# Autodesk Inventor assembly: ude_MIR
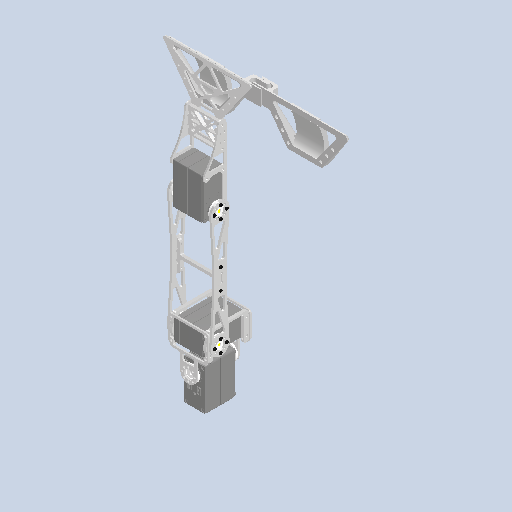
[picture p0: Inventor's stored thumbnail of the model, 512x512]
Saved by Autodesk Inventor 2024 (Build 280153000, 153)
## iProperties
Created: 2023-03-29
Part Number: ude_MIR
Document SubType Name: Assembly
Designer: right
Mass: 126.683 g
Surface Area: 569.35 cm^2
Volume: 110.135 cm^3
Density: 1.15025 g/cm^3
Author: right
## Documents named in this file (10)
- C:\Users\right\OneDrive\ドキュメント\Inventor\V2二足Light＿仮\ude_MIR.iam
- C:\Users\right\OneDrive\ドキュメント\Inventor\V2二足Light＿仮\KRS2500_scale_MIR1.ipt
- C:\Users\right\OneDrive\ドキュメント\Inventor\V2二足Light＿仮\02157_SmallDiameterHornB_MIR1.ipt
- C:\Users\right\OneDrive\ドキュメント\Inventor\V2二足Light＿仮\kata_MIR.ipt
- C:\Users\right\OneDrive\ドキュメント\Inventor\V2二足Light＿仮\腕_MIR.ipt
- C:\Users\right\OneDrive\ドキュメント\Inventor\V2二足Light＿仮\腕の筋交い_MIR.ipt
- C:\Users\right\OneDrive\ドキュメント\Inventor\V2二足Light＿仮\02159_SmallFreeHornC_MIR1.ipt
- C:\Users\right\OneDrive\ドキュメント\Inventor\V2二足Light＿仮\M2小ねじ_MIR.ipt
- C:\Users\right\OneDrive\ドキュメント\Inventor\V2二足Light＿仮\上腕_MIR.ipt
- C:\Users\right\OneDrive\ドキュメント\Inventor\V2二足Light＿仮\ヘラ.iam
## Components (41 placed, 9 different names)
1. KRS2500_scale_MIR1:1 — 挿入:1, 挿入:63, 角度:2
2. 02157_SmallDiameterHornB_MIR1:1 — 挿入:1, 挿入:5, 挿入:4
3. kata_MIR:1 — 挿入:5, 挿入:4, 挿入:56, 挿入:55, 挿入:54, 挿入:53, 挿入:67, 挿入:66, 挿入:71
4. KRS2500_scale_MIR1:2 — 挿入:10, 挿入:17, 挿入:70, 挿入:69, 挿入:74, 挿入:73
5. 02157_SmallDiameterHornB_MIR1:2 — 挿入:10, 挿入:16, 挿入:15
6. 腕_MIR:1 — 挿入:21, 挿入:20, 挿入:19, 挿入:18, 挿入:28, 挿入:27, 挿入:52, 挿入:48, 挿入:47, 挿入:49, 挿入:50, 挿入:46, 挿入:44, 挿入:45, 挿入:51, 挿入:43
7. 腕_MIR:2 — 挿入:16, 挿入:15, 挿入:22, 挿入:26, 挿入:25, 挿入:33, 挿入:37, 挿入:38, 挿入:40, 挿入:41, 挿入:35, 挿入:34, 挿入:36, 挿入:42, 挿入:39
8. 腕の筋交い_MIR:1 — 挿入:22, 挿入:21, 挿入:20, 角度:1, 角度:4
9. 02159_SmallFreeHornC_MIR1:1 — 挿入:19, 挿入:18, 挿入:17
10. KRS2500_scale_MIR1:3 — 挿入:23, 挿入:24
11. 02157_SmallDiameterHornB_MIR1:3 — 挿入:26, 挿入:25, 挿入:23
12. 02159_SmallFreeHornC_MIR1:2 — 挿入:28, 挿入:27, 挿入:24, 挿入:63
13. M2小ねじ_MIR:1 — 挿入:33
14. M2小ねじ_MIR:2 — 挿入:52
15. M2小ねじ_MIR:3 — 挿入:37
16. M2小ねじ_MIR:4 — 挿入:38
17. M2小ねじ_MIR:5 — 挿入:48
18. M2小ねじ_MIR:6 — 挿入:47
19. M2小ねじ_MIR:7 — 挿入:49
20. M2小ねじ_MIR:8 — 挿入:50
21. M2小ねじ_MIR:9 — 挿入:46
22. M2小ねじ_MIR:10 — 挿入:44
23. M2小ねじ_MIR:11 — 挿入:45
24. M2小ねじ_MIR:12 — 挿入:51
25. M2小ねじ_MIR:13 — 挿入:40
26. M2小ねじ_MIR:14 — 挿入:41
27. M2小ねじ_MIR:15 — 挿入:35
28. M2小ねじ_MIR:16 — 挿入:34
29. M2小ねじ_MIR:17 — 挿入:36
30. M2小ねじ_MIR:18 — 挿入:42
31. M2小ねじ_MIR:19 — 挿入:43
32. M2小ねじ_MIR:20 — 挿入:39
33. M2小ねじ_MIR:21 — 挿入:56
34. M2小ねじ_MIR:22 — 挿入:55
35. M2小ねじ_MIR:23 — 挿入:54
36. M2小ねじ_MIR:24 — 挿入:53
37. 02159_SmallFreeHornC_MIR1:3 — 挿入:63, 挿入:65, 挿入:64
38. kata_MIR:2 — 挿入:65, 挿入:64, 挿入:68, 挿入:72
39. 上腕_MIR:1 — 挿入:70, 挿入:69, 挿入:68, 挿入:67, 挿入:66
40. 上腕_MIR:2 — 挿入:74, 挿入:73, 挿入:72, 挿入:71, 角度:1, 角度:2
41. ヘラ:1 [sub-assembly] — 挿入:63, 角度:4
## Relationships (58: Insert 55, Angle 3)
- 挿入:1 [Insert]: KRS2500_scale_MIR1:1 ↔ 02157_SmallDiameterHornB_MIR1:1
- 挿入:5 [Insert]: 02157_SmallDiameterHornB_MIR1:1 ↔ kata_MIR:1
- 挿入:4 [Insert]: 02157_SmallDiameterHornB_MIR1:1 ↔ kata_MIR:1
- 挿入:10 [Insert]: KRS2500_scale_MIR1:2 ↔ 02157_SmallDiameterHornB_MIR1:2
- 挿入:16 [Insert]: 02157_SmallDiameterHornB_MIR1:2 ↔ 腕_MIR:2
- 挿入:15 [Insert]: 02157_SmallDiameterHornB_MIR1:2 ↔ 腕_MIR:2
- 挿入:22 [Insert]: 腕_MIR:2 ↔ 腕の筋交い_MIR:1
- 挿入:21 [Insert]: 腕_MIR:1 ↔ 腕の筋交い_MIR:1
- 挿入:20 [Insert]: 腕_MIR:1 ↔ 腕の筋交い_MIR:1
- 挿入:19 [Insert]: 腕_MIR:1 ↔ 02159_SmallFreeHornC_MIR1:1
- 挿入:18 [Insert]: 腕_MIR:1 ↔ 02159_SmallFreeHornC_MIR1:1
- 挿入:17 [Insert]: KRS2500_scale_MIR1:2 ↔ 02159_SmallFreeHornC_MIR1:1
- 挿入:26 [Insert]: 腕_MIR:2 ↔ 02157_SmallDiameterHornB_MIR1:3
- 挿入:25 [Insert]: 腕_MIR:2 ↔ 02157_SmallDiameterHornB_MIR1:3
- 挿入:23 [Insert]: KRS2500_scale_MIR1:3 ↔ 02157_SmallDiameterHornB_MIR1:3
- 挿入:28 [Insert]: 腕_MIR:1 ↔ 02159_SmallFreeHornC_MIR1:2
- 挿入:27 [Insert]: 腕_MIR:1 ↔ 02159_SmallFreeHornC_MIR1:2
- 挿入:24 [Insert]: KRS2500_scale_MIR1:3 ↔ 02159_SmallFreeHornC_MIR1:2
- 挿入:33 [Insert]: 腕_MIR:2 ↔ M2小ねじ_MIR:1
- 挿入:52 [Insert]: 腕_MIR:1 ↔ M2小ねじ_MIR:2
- 挿入:37 [Insert]: 腕_MIR:2 ↔ M2小ねじ_MIR:3
- 挿入:38 [Insert]: 腕_MIR:2 ↔ M2小ねじ_MIR:4
- 挿入:48 [Insert]: 腕_MIR:1 ↔ M2小ねじ_MIR:5
- 挿入:47 [Insert]: 腕_MIR:1 ↔ M2小ねじ_MIR:6
- 挿入:49 [Insert]: 腕_MIR:1 ↔ M2小ねじ_MIR:7
- 挿入:50 [Insert]: 腕_MIR:1 ↔ M2小ねじ_MIR:8
- 挿入:46 [Insert]: 腕_MIR:1 ↔ M2小ねじ_MIR:9
- 挿入:44 [Insert]: 腕_MIR:1 ↔ M2小ねじ_MIR:10
- 挿入:45 [Insert]: 腕_MIR:1 ↔ M2小ねじ_MIR:11
- 挿入:51 [Insert]: 腕_MIR:1 ↔ M2小ねじ_MIR:12
- 挿入:40 [Insert]: 腕_MIR:2 ↔ M2小ねじ_MIR:13
- 挿入:41 [Insert]: 腕_MIR:2 ↔ M2小ねじ_MIR:14
- 挿入:35 [Insert]: 腕_MIR:2 ↔ M2小ねじ_MIR:15
- 挿入:34 [Insert]: 腕_MIR:2 ↔ M2小ねじ_MIR:16
- 挿入:36 [Insert]: 腕_MIR:2 ↔ M2小ねじ_MIR:17
- 挿入:42 [Insert]: 腕_MIR:2 ↔ M2小ねじ_MIR:18
- 挿入:43 [Insert]: 腕_MIR:1 ↔ M2小ねじ_MIR:19
- 挿入:39 [Insert]: 腕_MIR:2 ↔ M2小ねじ_MIR:20
- 挿入:56 [Insert]: kata_MIR:1 ↔ M2小ねじ_MIR:21
- 挿入:55 [Insert]: kata_MIR:1 ↔ M2小ねじ_MIR:22
- 挿入:54 [Insert]: kata_MIR:1 ↔ M2小ねじ_MIR:23
- 挿入:53 [Insert]: kata_MIR:1 ↔ M2小ねじ_MIR:24
- 挿入:63 [Insert]: KRS2500_scale_MIR1:1 ↔ 02159_SmallFreeHornC_MIR1:3
- 挿入:65 [Insert]: 02159_SmallFreeHornC_MIR1:3 ↔ kata_MIR:2
- 挿入:64 [Insert]: 02159_SmallFreeHornC_MIR1:3 ↔ kata_MIR:2
- 挿入:70 [Insert]: KRS2500_scale_MIR1:2 ↔ 上腕_MIR:1
- 挿入:69 [Insert]: KRS2500_scale_MIR1:2 ↔ 上腕_MIR:1
- 挿入:68 [Insert]: kata_MIR:2 ↔ 上腕_MIR:1
- 挿入:67 [Insert]: kata_MIR:1 ↔ 上腕_MIR:1
- 挿入:66 [Insert]: kata_MIR:1 ↔ 上腕_MIR:1
- 挿入:74 [Insert]: KRS2500_scale_MIR1:2 ↔ 上腕_MIR:2
- 挿入:73 [Insert]: KRS2500_scale_MIR1:2 ↔ 上腕_MIR:2
- 挿入:72 [Insert]: kata_MIR:2 ↔ 上腕_MIR:2
- 挿入:71 [Insert]: kata_MIR:1 ↔ 上腕_MIR:2
- 角度:1 [Angle] (0 deg): 腕の筋交い_MIR:1 ↔ 上腕_MIR:2
- 角度:2 [Angle] (0 deg): KRS2500_scale_MIR1:1 ↔ 上腕_MIR:2
- 挿入:63 [Insert]: 02159_SmallFreeHornC_MIR1:2 ↔ ヘラ:1
- 角度:4 [Angle] (180 deg): 腕の筋交い_MIR:1 ↔ ヘラ:1
